# Autodesk Inventor assembly: Robot
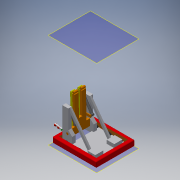
[picture p0: Inventor's stored thumbnail of the model, 180x180]
Saved by Autodesk Inventor 2016 (Build 200138000, 138)
## iProperties
Created: 2018-01-10
Part Number: Robot
Document SubType Name: Assembly
Designer: New User
Author: New User
## Documents named in this file (16)
- C:\Users\New User\Documents\Creations\2018\Robot.iam
- C:\Users\New User\Documents\Creations\2018\base.ipt
- C:\Users\New User\Documents\Creations\2018\elevbase.ipt
- C:\Users\New User\Documents\Creations\2018\cylendar.ipt
- C:\Users\New User\Documents\Creations\2018\piston.ipt
- C:\Users\New User\Documents\Creations\2018\elev1.ipt
- C:\Users\New User\Documents\Creations\2018\Slide.ipt
- C:\Users\New User\Documents\Creations\2018\arm.ipt
- C:\Users\New User\Documents\Creations\2018\arm2.ipt
- C:\Users\New User\Documents\Creations\2018\cylendar2.ipt
- C:\Users\New User\Documents\Creations\2018\piston2.ipt
- C:\Users\New User\Documents\Creations\2018\Robot\AIP\FEA\ce037cw00.fins
- C:\Users\New User\Documents\Creations\2018\Robot\AIP\FEA\ce037cw00.fsat
- C:\Users\New User\Documents\Creations\2018\Robot\AIP\FEA\ce037cw00.ftes
- C:\Users\New User\Documents\Creations\2018\Robot\AIP\FEA\ce037cw00.fwiz
- C:\Users\New User\Documents\Creations\2018\Robot\AIP\FEA\ce037cw80.fmsh
## Components (17 placed, 10 different names)
1. base:1 — Mate:1, Mate:2, Mate:4, Mate:5, Mate:8, Mate:9, Flush:7
2. elevbase:1 — Mate:1, Mate:2, Mate:6, Mate:10, Mate:11, Flush:3, Flush:5
3. cylendar:1 — Mate:3, Mate:4, Mate:5, Flush:1
4. piston:1 — Mate:3, Mate:6, Flush:1
5. cylendar:2 — Mate:8, Mate:9
6. piston:2 — Mate:10
7. elev1:1 — Mate:11, Flush:3, Mate:12, Flush:4, Flush:5, Flush:6
8. elev1:2 — Mate:12, Flush:4, Flush:6, Flush:9, Mate:13, Flush:10
9. Slide:1 — Flush:9, Mate:13, Flush:10, Mate:24, Mate:26, Mate:29, Mate:33, Flush:19
10. arm:2 — Mate:18, Mate:19, Mate:26, Angle:3, Flush:16, Mate:27, Flush:17, Flush:19, Flush:21
11. arm:3 — Flush:16, Mate:29, Mate:30, Flush:18, Mate:31, Mate:32, Angle:4, Flush:21
12. arm2:1 — Mate:31, Mate:32, Angle:4
13. arm2:2 — Mate:18, Mate:19, Angle:3
14. cylendar2:1 — Mate:22, Flush:13, Mate:24
15. piston2:1 — Mate:22, Flush:13, Mate:30, Flush:18
16. cylendar2:2 — Mate:33
17. piston2:2 — Mate:27, Flush:17
## Relationships (44: Mate 25, Flush 17, Angle 2)
- Mate:1: base:1 ↔ elevbase:1
- Mate:2: base:1 ↔ elevbase:1
- Mate:3: cylendar:1 ↔ piston:1
- Mate:4: base:1 ↔ cylendar:1
- Mate:5: base:1 ↔ cylendar:1
- Mate:6: elevbase:1 ↔ piston:1
- Flush:1: cylendar:1 ↔ piston:1
- [Mate]: cylendar:2 ↔ piston:2
- [Flush]: cylendar:2 ↔ piston:2
- Mate:8: base:1 ↔ cylendar:2
- Mate:9: base:1 ↔ cylendar:2
- Mate:10: elevbase:1 ↔ piston:2
- Mate:11: elevbase:1 ↔ elev1:1
- Flush:3: elevbase:1 ↔ elev1:1
- Mate:12: elev1:1 ↔ elev1:2
- Flush:4: elev1:1 ↔ elev1:2
- Flush:5: elevbase:1 ↔ elev1:1
- Flush:6: elev1:1 ↔ elev1:2
- Flush:7 (43.18 mm): base:1
- Flush:8 (-2133.6 mm)
- Flush:9: elev1:2 ↔ Slide:1
- Mate:13: elev1:2 ↔ Slide:1
- Flush:10: elev1:2 ↔ Slide:1
- Mate:18: arm:2 ↔ arm2:2
- Mate:19: arm:2 ↔ arm2:2
- Mate:22: cylendar2:1 ↔ piston2:1
- Flush:13: cylendar2:1 ↔ piston2:1
- Mate:24: Slide:1 ↔ cylendar2:1
- [Mate]: cylendar2:2 ↔ piston2:2
- [Flush]: cylendar2:2 ↔ piston2:2
- Mate:26: Slide:1 ↔ arm:2
- Angle:3 (-99 deg): arm:2 ↔ arm2:2
- Flush:16: arm:2 ↔ arm:3
- Mate:27: arm:2 ↔ piston2:2
- Flush:17: arm:2 ↔ piston2:2
- Mate:29: Slide:1 ↔ arm:3
- Mate:30: arm:3 ↔ piston2:1
- Flush:18: arm:3 ↔ piston2:1
- Mate:31: arm:3 ↔ arm2:1
- Mate:32: arm:3 ↔ arm2:1
- Angle:4 (-99 deg): arm:3 ↔ arm2:1
- Mate:33: Slide:1 ↔ cylendar2:2
- Flush:19: Slide:1 ↔ arm:2
- Flush:21: arm:2 ↔ arm:3
## Named parameters: d40_d37 = 0 mm, d41_d38 = 266.7 mm, d42_d39 = 0 mm, d43_d20 = 0 mm, d100_d89 = 0 mm, d101_d95 = 0 mm, d102_d96 = 40.64 mm, d103_d97 = 0 mm
